# Autodesk Inventor assembly: IntakeSlides2.0
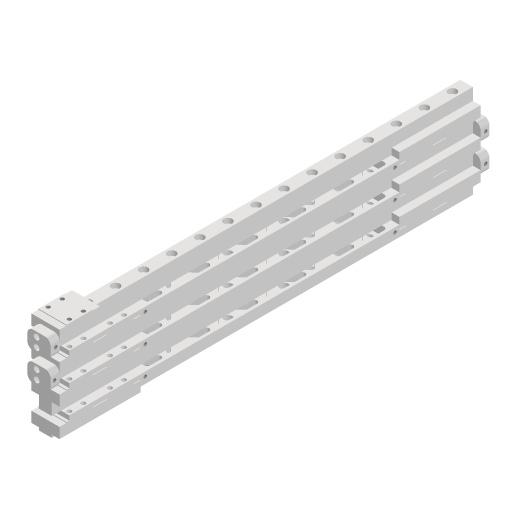
[picture p0: Inventor's stored thumbnail of the model, 512x512]
Saved by Autodesk Inventor 2023 (Build 270158000, 158)
## iProperties
Created: 2022-09-16
Part Number: IntakeSlides2.0
Document SubType Name: Assembly
Designer: deli
Author: deli
## Documents named in this file (5)
- C:\Users\deli\OneDrive - Eastside Preparatory School\FTC\8103-power-play\CAD\IntakeSlides2.0.iam
- C:\Users\deli\OneDrive - Eastside Preparatory School\FTC\8103-power-play\CAD\SlideStopBearingHolder.ipt
- C:\Users\deli\OneDrive - Eastside Preparatory School\FTC\8103-power-play\CAD\Rail.ipt
- C:\Users\deli\OneDrive - Eastside Preparatory School\FTC\8103-power-play\CAD\Carrige.ipt
- C:\Users\deli\OneDrive - Eastside Preparatory School\FTC\8103-power-play\CAD\Connector Plate.ipt
## Components (28 placed, 4 different names)
1. SlideStopBearingHolder:1 — Mate:72, Mate:73, Mate:74
2. SlideStopBearingHolder:2 — Mate:67, Mate:68, Mate:85
3. SlideStopBearingHolder:4 — Mate:69, Mate:70, Mate:71
4. Rail:1 — Mate:61, Flush:16, Flush:17, Mate:69, Mate:71, Mate:78, Mate:80
5. Carrige:1
6. Carrige:2
7. Carrige:3
8. Carrige:4 — Flush:22
9. Connector Plate:1
10. Rail:2 — Mate:65, Flush:19, Flush:20, Mate:72, Mate:73, Flush:22
11. Rail:3 — Mate:60, Flush:14, Flush:15, Mate:67, Mate:81, Mate:83
12. Carrige:5 — Mate:85
13. Carrige:6
14. Carrige:7
15. Carrige:8 — Mate:88
16. Connector Plate:2
17. Rail:4 — Mate:61, Flush:16, Flush:17, Mate:70, Mate:79
18. Rail:5
19. Carrige:9
20. Carrige:10
21. Carrige:11
22. Carrige:12 — Mate:84
23. Connector Plate:3
24. Rail:6 — Mate:60, Flush:14, Flush:15, Mate:68, Mate:82
25. Carrige:14 — Flush:21
26. Rail:7 — Mate:65, Flush:19, Flush:20, Mate:74, Flush:21
27. SlideStopBearingHolder:5 — Mate:78, Mate:79, Mate:80, Mate:88
28. SlideStopBearingHolder:6 — Mate:81, Mate:82, Mate:83, Mate:84
## Relationships (81: Mate 67, Flush 14)
- [Mate]: Rail:1 ↔ Carrige:2
- [Mate]: Rail:1 ↔ Carrige:1
- [Mate]: Rail:1 ↔ Carrige:1
- [Mate]: Rail:1 ↔ Carrige:2
- [Mate]: Carrige:1 ↔ Carrige:2
- [Mate]: Carrige:3 ↔ Carrige:4
- [Mate]: Carrige:4 ↔ Rail:2
- [Mate]: Carrige:4 ↔ Rail:2
- [Flush]: Carrige:3 ↔ Carrige:4
- [Mate]: Carrige:1 ↔ Connector Plate:1
- [Mate]: Carrige:1 ↔ Connector Plate:1
- [Mate]: Carrige:1 ↔ Connector Plate:1
- [Mate]: Carrige:3 ↔ Connector Plate:1
- [Mate]: Carrige:3 ↔ Connector Plate:1
- [Mate]: Carrige:4 ↔ Connector Plate:1
- [Mate]: Carrige:4 ↔ Connector Plate:1
- [Flush]: Rail:1 ↔ Carrige:1
- [Mate]: Rail:3 ↔ Carrige:6
- [Mate]: Rail:3 ↔ Carrige:5
- [Mate]: Rail:3 ↔ Carrige:5
- [Mate]: Rail:3 ↔ Carrige:6
- [Mate]: Carrige:5 ↔ Carrige:6
- [Mate]: Carrige:7 ↔ Carrige:8
- [Mate]: Carrige:8 ↔ Rail:4
- [Mate]: Carrige:8 ↔ Rail:4
- [Flush]: Carrige:7 ↔ Carrige:8
- [Mate]: Carrige:5 ↔ Connector Plate:2
- [Mate]: Carrige:5 ↔ Connector Plate:2
- [Mate]: Carrige:5 ↔ Connector Plate:2
- [Mate]: Carrige:7 ↔ Connector Plate:2
- [Mate]: Carrige:7 ↔ Connector Plate:2
- [Mate]: Carrige:8 ↔ Connector Plate:2
- [Mate]: Carrige:8 ↔ Connector Plate:2
- [Flush]: Rail:3 ↔ Carrige:5
- [Mate]: Rail:5 ↔ Carrige:10
- [Mate]: Rail:5 ↔ Carrige:9
- [Mate]: Rail:5 ↔ Carrige:9
- [Mate]: Rail:5 ↔ Carrige:10
- [Mate]: Carrige:9 ↔ Carrige:10
- [Mate]: Carrige:11 ↔ Carrige:12
- [Mate]: Carrige:12 ↔ Rail:6
- [Mate]: Carrige:12 ↔ Rail:6
- [Flush]: Carrige:11 ↔ Carrige:12
- [Mate]: Carrige:9 ↔ Connector Plate:3
- [Mate]: Carrige:9 ↔ Connector Plate:3
- [Mate]: Carrige:9 ↔ Connector Plate:3
- [Mate]: Carrige:11 ↔ Connector Plate:3
- [Mate]: Carrige:11 ↔ Connector Plate:3
- [Mate]: Carrige:12 ↔ Connector Plate:3
- [Mate]: Carrige:12 ↔ Connector Plate:3
- [Flush]: Rail:5 ↔ Carrige:9
- Mate:60: Rail:3 ↔ Rail:6
- Flush:14: Rail:3 ↔ Rail:6
- Flush:15: Rail:3 ↔ Rail:6
- Mate:61: Rail:1 ↔ Rail:4
- Flush:16: Rail:1 ↔ Rail:4
- Flush:17: Rail:1 ↔ Rail:4
- [Mate]: Carrige:14 ↔ Rail:7
- [Mate]: Carrige:14 ↔ Rail:7
- Mate:65: Rail:2 ↔ Rail:7
- Flush:19: Rail:2 ↔ Rail:7
- Flush:20: Rail:2 ↔ Rail:7
- Mate:67: SlideStopBearingHolder:2 ↔ Rail:3
- Mate:68: SlideStopBearingHolder:2 ↔ Rail:6
- Mate:69: SlideStopBearingHolder:4 ↔ Rail:1
- Mate:70: SlideStopBearingHolder:4 ↔ Rail:4
- Mate:71: SlideStopBearingHolder:4 ↔ Rail:1
- Mate:72: SlideStopBearingHolder:1 ↔ Rail:2
- Mate:73: SlideStopBearingHolder:1 ↔ Rail:2
- Mate:74: SlideStopBearingHolder:1 ↔ Rail:7
- Mate:78: Rail:1 ↔ SlideStopBearingHolder:5
- Mate:79: Rail:4 ↔ SlideStopBearingHolder:5
- Mate:80: Rail:1 ↔ SlideStopBearingHolder:5
- Mate:81: Rail:3 ↔ SlideStopBearingHolder:6
- Mate:82: Rail:6 ↔ SlideStopBearingHolder:6
- Mate:83: Rail:3 ↔ SlideStopBearingHolder:6
- Mate:84: Carrige:12 ↔ SlideStopBearingHolder:6
- Mate:85: SlideStopBearingHolder:2 ↔ Carrige:5
- Mate:88: Carrige:8 ↔ SlideStopBearingHolder:5
- Flush:21 (-271.1 mm): Carrige:14 ↔ Rail:7
- Flush:22: Carrige:4 ↔ Rail:2
## Named parameters: d35_d20 = 0 mm, stroke = 0 mm, d49_d4 = 0 mm, d50_d5 = 0 mm, d51_d6 = 0 mm, d52_d7 = 0 mm, d53_d8 = 0 mm, d54_d20 = 0 mm, d55_d77 = 0 mm, d56_d78 = 0 mm, d57_d83 = 0 mm, d58_d86 = 0 mm, d59_d87 = 0 mm, d60_d88 = 0 mm, d61_d89 = 0 mm, d62_d90 = 0 mm, d63_d91 = 0 mm, d64_d92 = 0 mm, d67_d112 = 0 mm, d68_d4 = 0 mm, d69_d5 = 0 mm, d70_d6 = 0 mm, d71_d7 = 0 mm, d72_d8 = 0 mm, d73_d20 = 0 mm, d74_d77 = 0 mm, d75_d78 = 0 mm, d76_d83 = 0 mm, d79_d86 = 0 mm, d80_d87 = 0 mm, d81_d88 = 0 mm, d82_d89 = 0 mm, d84_d90 = 0 mm, d85_d91 = 0 mm, d93_d92 = 0 mm, d96_d112 = 0 mm, d104_d77 = 0 mm, d105_d78 = 0 mm
